# Autodesk Inventor assembly: Battery_Mount_2Cell_Assembled_V1
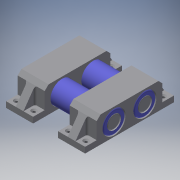
[picture p0: Inventor's stored thumbnail of the model, 180x180]
Saved by Autodesk Inventor 2016 (Build 200138000, 138)
## iProperties
Created: 2016-11-21
Part Number: Battery_Mount_2Cell_Assembled_V1
Document SubType Name: Assembly
Designer: Christopher
Author: Christopher
## Documents named in this file (3)
- C:\Users\Pierce\Documents\College\CACTUS I\CADD\HERMES\CADD\Battery_Mount_2Cell_Assembled_V1.iam
- C:\Users\Pierce\Documents\College\CACTUS I\CADD\HERMES\CADD\18650_thmjpr.ipt
- C:\Users\Pierce\Documents\College\CACTUS I\CADD\HERMES\CADD\Battery_Mount_1U_Hermes_V1.ipt
## Components (4 placed, 2 different names)
1. 18650_thmjpr:1 — Mate:1, Flush:1, Mate:4, Flush:2
2. Battery_Mount_1U_Hermes_V1:1 — Mate:1, Flush:1, Mate:2, Mate:3
3. 18650_thmjpr:2 — Mate:2, Mate:3, Mate:5
4. Battery_Mount_1U_Hermes_V1:2 — Mate:4, Flush:2, Mate:5
## Relationships (7: Mate 5, Flush 2)
- Mate:1: 18650_thmjpr:1 ↔ Battery_Mount_1U_Hermes_V1:1
- Flush:1: 18650_thmjpr:1 ↔ Battery_Mount_1U_Hermes_V1:1
- Mate:2: Battery_Mount_1U_Hermes_V1:1 ↔ 18650_thmjpr:2
- Mate:3: Battery_Mount_1U_Hermes_V1:1 ↔ 18650_thmjpr:2
- Mate:4: 18650_thmjpr:1 ↔ Battery_Mount_1U_Hermes_V1:2
- Flush:2: 18650_thmjpr:1 ↔ Battery_Mount_1U_Hermes_V1:2
- Mate:5: 18650_thmjpr:2 ↔ Battery_Mount_1U_Hermes_V1:2
